# Autodesk Inventor assembly: chain_MIR
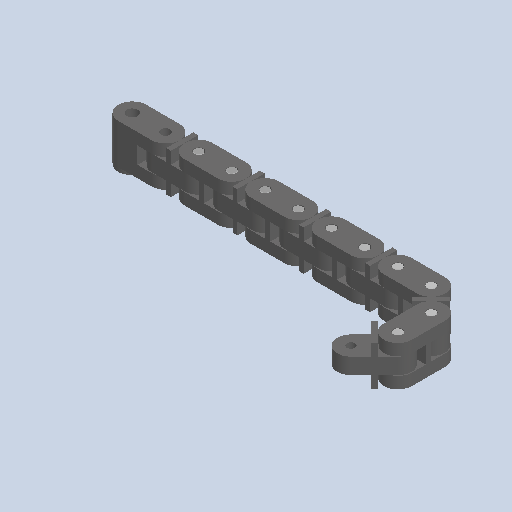
[picture p0: Inventor's stored thumbnail of the model, 512x512]
Saved by Autodesk Inventor 2024.1 (Build 281209000, 209)
## iProperties
Created: 2025-01-18
Part Number: chain_MIR
Document SubType Name: Assembly
Designer: hibik
Author: hibik
## Documents named in this file (5)
- C:\Users\hibik\Documents\Robomech\RESCUE\ORCA\hard\fork\right\chain_MIR.iam
- C:\Users\hibik\Documents\Robomech\RESCUE\ORCA\hard\fork\right\chain_2_MIR.ipt
- C:\Users\hibik\Documents\Robomech\RESCUE\ORCA\hard\fork\right\chain_1_MIR.ipt
- C:\Users\hibik\Documents\Robomech\RESCUE\ORCA\hard\std_parts\shaft_2_10_MIR.ipt
- C:\Users\hibik\Documents\Robomech\RESCUE\ORCA\hard\fork\right\chain_fork_connector_MIR.ipt
## Components (22 placed, 4 different names)
1. chain_2_MIR:1 — メイト:1, 角度:8, フラッシュ:12, 角度:4, 挿入:9
2. chain_1_MIR:1 — 角度:4, 挿入:9, 挿入:10, 角度:5, 挿入:24, 挿入:32
3. shaft_2_10_MIR:1 — 挿入:10
4. chain_2_MIR:2 — 角度:5, 挿入:24, 角度:6, 挿入:11
5. chain_1_MIR:2 — 角度:6, 挿入:11, 挿入:12, 角度:7, 挿入:25, フラッシュ:5, 挿入:33
6. shaft_2_10_MIR:2 — 挿入:12
7. chain_2_MIR:3 — 角度:7, 挿入:25, 挿入:13, フラッシュ:6
8. chain_1_MIR:3 — フラッシュ:5, 挿入:13, 挿入:14, 挿入:26, フラッシュ:7, 挿入:34
9. shaft_2_10_MIR:3 — 挿入:14
10. chain_2_MIR:4 — フラッシュ:6, 挿入:26, 挿入:15, フラッシュ:8
11. chain_1_MIR:4 — フラッシュ:7, 挿入:15, 挿入:16, 挿入:27, フラッシュ:9, 挿入:35
12. shaft_2_10_MIR:4 — 挿入:16
13. chain_2_MIR:5 — フラッシュ:8, 挿入:27, 挿入:17, フラッシュ:10
14. chain_1_MIR:5 — フラッシュ:9, 挿入:17, 挿入:18, 挿入:28, 挿入:36, フラッシュ:13
15. shaft_2_10_MIR:5 — 挿入:18
16. chain_2_MIR:6 — フラッシュ:10, 挿入:28, 挿入:37
17. shaft_2_10_MIR:6 — 挿入:32
18. shaft_2_10_MIR:7 — 挿入:33
19. shaft_2_10_MIR:8 — 挿入:34
20. shaft_2_10_MIR:9 — 挿入:35
21. shaft_2_10_MIR:10 — 挿入:36
22. chain_fork_connector_MIR:1 — フラッシュ:13, 挿入:37
## Relationships (35: Insert 21, Flush 8, Angle 5, Mate 1)
- メイト:1 [Mate]: chain_2_MIR:1
- 角度:8 [Angle] (45 deg): chain_2_MIR:1
- フラッシュ:12 [Flush]: chain_2_MIR:1
- 角度:4 [Angle] (-45 deg): chain_2_MIR:1 ↔ chain_1_MIR:1
- 挿入:9 [Insert] (0.1 mm): chain_2_MIR:1 ↔ chain_1_MIR:1
- 挿入:10 [Insert]: chain_1_MIR:1 ↔ shaft_2_10_MIR:1
- 角度:5 [Angle] (-45 deg): chain_1_MIR:1 ↔ chain_2_MIR:2
- 挿入:24 [Insert] (0.1 mm): chain_1_MIR:1 ↔ chain_2_MIR:2
- 角度:6 [Angle] (-45 deg): chain_2_MIR:2 ↔ chain_1_MIR:2
- 挿入:11 [Insert] (0.1 mm): chain_2_MIR:2 ↔ chain_1_MIR:2
- 挿入:12 [Insert]: chain_1_MIR:2 ↔ shaft_2_10_MIR:2
- 角度:7 [Angle] (0 deg): chain_1_MIR:2 ↔ chain_2_MIR:3
- 挿入:25 [Insert] (0.1 mm): chain_1_MIR:2 ↔ chain_2_MIR:3
- フラッシュ:5 [Flush]: chain_1_MIR:2 ↔ chain_1_MIR:3
- 挿入:13 [Insert] (0.1 mm): chain_2_MIR:3 ↔ chain_1_MIR:3
- 挿入:14 [Insert]: chain_1_MIR:3 ↔ shaft_2_10_MIR:3
- フラッシュ:6 [Flush]: chain_2_MIR:3 ↔ chain_2_MIR:4
- 挿入:26 [Insert] (0.1 mm): chain_1_MIR:3 ↔ chain_2_MIR:4
- フラッシュ:7 [Flush]: chain_1_MIR:3 ↔ chain_1_MIR:4
- 挿入:15 [Insert] (0.1 mm): chain_2_MIR:4 ↔ chain_1_MIR:4
- 挿入:16 [Insert]: chain_1_MIR:4 ↔ shaft_2_10_MIR:4
- フラッシュ:8 [Flush]: chain_2_MIR:4 ↔ chain_2_MIR:5
- 挿入:27 [Insert] (0.1 mm): chain_1_MIR:4 ↔ chain_2_MIR:5
- フラッシュ:9 [Flush]: chain_1_MIR:4 ↔ chain_1_MIR:5
- 挿入:17 [Insert] (0.1 mm): chain_2_MIR:5 ↔ chain_1_MIR:5
- 挿入:18 [Insert]: chain_1_MIR:5 ↔ shaft_2_10_MIR:5
- フラッシュ:10 [Flush]: chain_2_MIR:5 ↔ chain_2_MIR:6
- 挿入:28 [Insert] (0.1 mm): chain_1_MIR:5 ↔ chain_2_MIR:6
- 挿入:32 [Insert]: chain_1_MIR:1 ↔ shaft_2_10_MIR:6
- 挿入:33 [Insert]: chain_1_MIR:2 ↔ shaft_2_10_MIR:7
- 挿入:34 [Insert]: chain_1_MIR:3 ↔ shaft_2_10_MIR:8
- 挿入:35 [Insert]: chain_1_MIR:4 ↔ shaft_2_10_MIR:9
- 挿入:36 [Insert]: chain_1_MIR:5 ↔ shaft_2_10_MIR:10
- フラッシュ:13 [Flush]: chain_1_MIR:5 ↔ chain_fork_connector_MIR:1
- 挿入:37 [Insert] (0.1 mm): chain_2_MIR:6 ↔ chain_fork_connector_MIR:1
